# Autodesk Inventor assembly: SpoolHolder
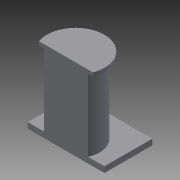
[picture p0: Inventor's stored thumbnail of the model, 180x180]
Saved by Autodesk Inventor 2015 SP1 (Build 190203100, 203)
## iProperties
Created: 2015-04-19
Part Number: SpoolHolder
Document SubType Name: Assembly
Designer: Jack
Author: Jack
## Documents named in this file (4)
- C:\Users\Jack\ownCloud\Projects\CrossBot\InventorModel\Enclosure\SpoolHolder\SpoolHolder.iam
- C:\Users\Jack\ownCloud\Projects\CrossBot\InventorModel\Enclosure\SpoolHolder\SpoolHolderSingle.ipt
- C:\Users\Jack\ownCloud\Projects\CrossBot\InventorModel\Hardware\Bearing\BearingRadialBall\BearingRadialBall608zz.ipt
- C:\Users\Jack\ownCloud\Projects\CrossBot\InventorModel\Enclosure\SpoolHolder\SpoolHolderBearingShaft.ipt
## Components (5 placed, 3 different names)
1. SpoolHolderSingle:1 — Mate:1, Mate:2, Mate:3, Mate:4, Mate:6, Mate:8
2. BearingRadialBall608zz:1 — Mate:5, Mate:6
3. BearingRadialBall608zz:2 — Mate:7, Mate:8
4. SpoolHolderBearingShaft:1 — Mate:1, Mate:2, Mate:5
5. SpoolHolderBearingShaft:2 — Mate:3, Mate:4, Mate:7
## Relationships (8: Mate 8)
- Mate:1: SpoolHolderSingle:1 ↔ SpoolHolderBearingShaft:1
- Mate:2: SpoolHolderSingle:1 ↔ SpoolHolderBearingShaft:1
- Mate:3: SpoolHolderSingle:1 ↔ SpoolHolderBearingShaft:2
- Mate:4: SpoolHolderSingle:1 ↔ SpoolHolderBearingShaft:2
- Mate:5: BearingRadialBall608zz:1 ↔ SpoolHolderBearingShaft:1
- Mate:6 (0.25 mm): SpoolHolderSingle:1 ↔ BearingRadialBall608zz:1
- Mate:7: BearingRadialBall608zz:2 ↔ SpoolHolderBearingShaft:2
- Mate:8 (0.25 mm): SpoolHolderSingle:1 ↔ BearingRadialBall608zz:2
